# Autodesk Inventor assembly: Omniwheel (ME)
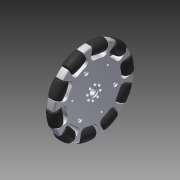
[picture p0: Inventor's stored thumbnail of the model, 180x180]
Saved by Autodesk Inventor 2015 (Build 190159000, 159)
## iProperties
Created: 2016-10-07
Part Number: Omniwheel (ME)
Document SubType Name: Assembly
Designer: Mason
Author: Mason
## Documents named in this file (3)
- C:\Users\User\Documents\Inventor\Content Center Files\FTC\Wheels\Omniwheel (ME).iam
- C:\Users\User\Documents\Inventor\Content Center Files\FTC\MAX Omniwheel parts\Roller ASM parts\Roller 736466\tetrix_736466_roller.iam
- C:\Users\User\Documents\Inventor\Content Center Files\FTC\MAX Omniwheel parts\tetrix_736466_hub.ipt
## Components (12 placed, 2 different names)
1. tetrix_736466_hub:1 — Mate:1, Mate:2, Flush:1, Mate:4, Mate:5
2. tetrix_736466_hub:2 — Mate:1, Mate:2, Flush:1, Mate:3
3. tetrix_736466_roller:2 [sub-assembly] — Mate:3, Mate:4, Mate:5
4. tetrix_736466_roller:3 [sub-assembly]
5. tetrix_736466_roller:4 [sub-assembly]
6. tetrix_736466_roller:5 [sub-assembly]
7. tetrix_736466_roller:6 [sub-assembly]
8. tetrix_736466_roller:7 [sub-assembly]
9. tetrix_736466_roller:8 [sub-assembly]
10. tetrix_736466_roller:9 [sub-assembly]
11. tetrix_736466_roller:10 [sub-assembly]
12. tetrix_736466_roller:11 [sub-assembly]
## Component patterns: (10 elements, first: tetrix_736466_roller:2)
## Relationships (6: Mate 5, Flush 1)
- Mate:1: tetrix_736466_hub:1 ↔ tetrix_736466_hub:2
- Mate:2: tetrix_736466_hub:1 ↔ tetrix_736466_hub:2
- Flush:1: tetrix_736466_hub:1 ↔ tetrix_736466_hub:2
- Mate:3: tetrix_736466_hub:2 ↔ tetrix_736466_roller:2
- Mate:4: tetrix_736466_hub:1 ↔ tetrix_736466_roller:2
- Mate:5: tetrix_736466_hub:1 ↔ tetrix_736466_roller:2
